# Autodesk Inventor assembly: BG101_trajan20_22
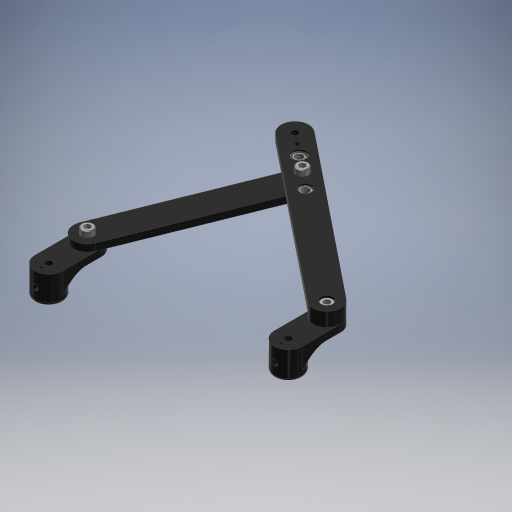
[picture p0: Inventor's stored thumbnail of the model, 512x512]
Saved by Autodesk Inventor 2023 (Build 270158000, 158)
## iProperties
Company: HTBLA Kaindorf
RuleStatus: InUse
Created: 2022-11-06
Part Number: BG101_trajan20_22
Project: Zeichenmaschine_neu
Material: Generisch
Description: Gelenke
Document SubType Name: Assembly
Designer: trajan20
AfterDocNew0: iProperties-Editor_aufrufen
Author: jan
Keywords: 2022
## Documents named in this file (9)
- C:\Users\jan\Documents\Zeichenmaschine_neu\BG101_trajan20_22_Zeichenmaschine_neu_Gelenke.iam
- C:\Users\jan\Documents\Zeichenmaschine_neu\BT301_trajan20_21_Zeichenmaschine_v2_gelenk 1.ipt
- C:\Users\jan\Documents\Zeichenmaschine_neu\BT301_trajan20_21_Zeichenmaschine_v2_gelenk a.ipt
- C:\Users\jan\Documents\Zeichenmaschine_neu\BT303_trajan20_21_Zeichenmaschine_v2_gelenk b.ipt
- C:\Users\jan\Documents\Zeichenmaschine_neu\eigene Normteile\DIN 625 SKF - SKF 628_5-2Z_5x10x4.ipt
- C:\Users\jan\Documents\Zeichenmaschine_neu\Normteile\de-DE\ISO 4762(2)\ISO 4762 - M5 x 16ISO.ipt
- C:\Users\jan\Documents\Zeichenmaschine_neu\Normteile\de-DE\ISO 10511\ISO 10511 - M5.ipt
- C:\Users\jan\Documents\Zeichenmaschine_neu\Normteile\de-DE\DIN 916\DIN 916 - M4  x  10.ipt
- C:\Users\jan\Documents\Zeichenmaschine_neu\BT004_trajan20_22_Zeichenmaschine_neu_QuadratMutter.ipt
## Components (19 placed, 8 different names)
1. BT301_trajan20_21_Zeichenmaschine_v2_gelenk 1:1 — Fluchtend:1, Passend:18, Passend:19, Passend:32, Passend:35, Passend:40, Passend:43, Winkel:1, Passend:45, Passend:46
2. BT301_trajan20_21_Zeichenmaschine_v2_gelenk 1:2 — Fluchtend:1, Passend:4, Passend:5, Passend:30, Passend:37, Passend:41, Passend:43, Winkel:2, Passend:47, Passend:48
3. BT301_trajan20_21_Zeichenmaschine_v2_gelenk a:1 — Passend:18, Passend:19, Passend:20, Passend:21, Passend:22, Passend:34
4. BT303_trajan20_21_Zeichenmaschine_v2_gelenk b:1 — Passend:4, Passend:5, Passend:8, Passend:9, Passend:10, Passend:11, Passend:12, Passend:13, Passend:16, Passend:17, Passend:44
5. BT004_trajan20_22_Zeichenmaschine_neu_QuadratMutter:1 — Winkel:1, Passend:45, Passend:46
6. BT004_trajan20_22_Zeichenmaschine_neu_QuadratMutter:2 — Winkel:2, Passend:47, Passend:48
7. DIN 625 SKF- beidseitig abgedeckt SKF 628/5-2Z:1 — Passend:8, Passend:9
8. DIN 625 SKF- beidseitig abgedeckt SKF 628/5-2Z:2 — Passend:10, Passend:11, Passend:22, Passend:25, Passend:26
9. DIN 625 SKF- beidseitig abgedeckt SKF 628/5-2Z:3 — Passend:12, Passend:13
10. DIN 625 SKF- beidseitig abgedeckt SKF 628/5-2Z:4 — Passend:20, Passend:21, Passend:23, Passend:24
11. DIN 625 SKF- beidseitig abgedeckt SKF 628/5-2Z:5 — Passend:16, Passend:17, Passend:27, Passend:28
12. ISO 4762 M5 x 16:1 — Passend:23, Passend:24, Passend:31, Passend:44
13. ISO 4762 M5 x 16:2 — Passend:25, Passend:26, Passend:33
14. ISO 4762 M5 x 16:3 — Passend:27, Passend:28, Passend:29
15. DIN EN ISO 10511 M5:1 — Passend:29, Passend:30
16. DIN EN ISO 10511 M5:2 — Passend:31, Passend:32
17. DIN EN ISO 10511 M5:3 — Passend:33, Passend:34
18. DIN 916 M4  x  10:1 — Passend:35, Passend:40
19. DIN 916 M4  x  10:3 — Passend:37, Passend:41
## Relationships (40: Mate 37, Angle 2, Flush 1)
- Fluchtend:1 [Flush]: BT301_trajan20_21_Zeichenmaschine_v2_gelenk 1:1 ↔ BT301_trajan20_21_Zeichenmaschine_v2_gelenk 1:2
- Passend:4 [Mate]: BT301_trajan20_21_Zeichenmaschine_v2_gelenk 1:2 ↔ BT303_trajan20_21_Zeichenmaschine_v2_gelenk b:1
- Passend:5 [Mate]: BT301_trajan20_21_Zeichenmaschine_v2_gelenk 1:2 ↔ BT303_trajan20_21_Zeichenmaschine_v2_gelenk b:1
- Passend:8 [Mate]: BT303_trajan20_21_Zeichenmaschine_v2_gelenk b:1 ↔ DIN 625 SKF- beidseitig abgedeckt SKF 628/5-2Z:1
- Passend:9 [Mate]: BT303_trajan20_21_Zeichenmaschine_v2_gelenk b:1 ↔ DIN 625 SKF- beidseitig abgedeckt SKF 628/5-2Z:1
- Passend:10 [Mate]: BT303_trajan20_21_Zeichenmaschine_v2_gelenk b:1 ↔ DIN 625 SKF- beidseitig abgedeckt SKF 628/5-2Z:2
- Passend:11 [Mate]: BT303_trajan20_21_Zeichenmaschine_v2_gelenk b:1 ↔ DIN 625 SKF- beidseitig abgedeckt SKF 628/5-2Z:2
- Passend:12 [Mate]: BT303_trajan20_21_Zeichenmaschine_v2_gelenk b:1 ↔ DIN 625 SKF- beidseitig abgedeckt SKF 628/5-2Z:3
- Passend:13 [Mate]: BT303_trajan20_21_Zeichenmaschine_v2_gelenk b:1 ↔ DIN 625 SKF- beidseitig abgedeckt SKF 628/5-2Z:3
- Passend:16 [Mate]: BT303_trajan20_21_Zeichenmaschine_v2_gelenk b:1 ↔ DIN 625 SKF- beidseitig abgedeckt SKF 628/5-2Z:5
- Passend:17 [Mate]: BT303_trajan20_21_Zeichenmaschine_v2_gelenk b:1 ↔ DIN 625 SKF- beidseitig abgedeckt SKF 628/5-2Z:5
- Passend:18 [Mate]: BT301_trajan20_21_Zeichenmaschine_v2_gelenk 1:1 ↔ BT301_trajan20_21_Zeichenmaschine_v2_gelenk a:1
- Passend:19 [Mate]: BT301_trajan20_21_Zeichenmaschine_v2_gelenk 1:1 ↔ BT301_trajan20_21_Zeichenmaschine_v2_gelenk a:1
- Passend:20 [Mate]: BT301_trajan20_21_Zeichenmaschine_v2_gelenk a:1 ↔ DIN 625 SKF- beidseitig abgedeckt SKF 628/5-2Z:4
- Passend:21 [Mate]: BT301_trajan20_21_Zeichenmaschine_v2_gelenk a:1 ↔ DIN 625 SKF- beidseitig abgedeckt SKF 628/5-2Z:4
- Passend:22 [Mate]: BT301_trajan20_21_Zeichenmaschine_v2_gelenk a:1 ↔ DIN 625 SKF- beidseitig abgedeckt SKF 628/5-2Z:2
- Passend:23 [Mate]: DIN 625 SKF- beidseitig abgedeckt SKF 628/5-2Z:4 ↔ ISO 4762 M5 x 16:1
- Passend:24 [Mate]: DIN 625 SKF- beidseitig abgedeckt SKF 628/5-2Z:4 ↔ ISO 4762 M5 x 16:1
- Passend:25 [Mate]: DIN 625 SKF- beidseitig abgedeckt SKF 628/5-2Z:2 ↔ ISO 4762 M5 x 16:2
- Passend:26 [Mate]: DIN 625 SKF- beidseitig abgedeckt SKF 628/5-2Z:2 ↔ ISO 4762 M5 x 16:2
- Passend:27 [Mate]: DIN 625 SKF- beidseitig abgedeckt SKF 628/5-2Z:5 ↔ ISO 4762 M5 x 16:3
- Passend:28 [Mate]: DIN 625 SKF- beidseitig abgedeckt SKF 628/5-2Z:5 ↔ ISO 4762 M5 x 16:3
- Passend:29 [Mate]: ISO 4762 M5 x 16:3 ↔ DIN EN ISO 10511 M5:1
- Passend:30 [Mate]: BT301_trajan20_21_Zeichenmaschine_v2_gelenk 1:2 ↔ DIN EN ISO 10511 M5:1
- Passend:31 [Mate]: ISO 4762 M5 x 16:1 ↔ DIN EN ISO 10511 M5:2
- Passend:32 [Mate]: BT301_trajan20_21_Zeichenmaschine_v2_gelenk 1:1 ↔ DIN EN ISO 10511 M5:2
- Passend:33 [Mate]: ISO 4762 M5 x 16:2 ↔ DIN EN ISO 10511 M5:3
- Passend:34 [Mate]: BT301_trajan20_21_Zeichenmaschine_v2_gelenk a:1 ↔ DIN EN ISO 10511 M5:3
- Passend:35 [Mate]: BT301_trajan20_21_Zeichenmaschine_v2_gelenk 1:1 ↔ DIN 916 M4  x  10:1
- Passend:37 [Mate]: BT301_trajan20_21_Zeichenmaschine_v2_gelenk 1:2 ↔ DIN 916 M4  x  10:3
- Passend:40 [Mate]: BT301_trajan20_21_Zeichenmaschine_v2_gelenk 1:1 ↔ DIN 916 M4  x  10:1
- Passend:41 [Mate]: BT301_trajan20_21_Zeichenmaschine_v2_gelenk 1:2 ↔ DIN 916 M4  x  10:3
- Passend:43 [Mate] (140 mm): BT301_trajan20_21_Zeichenmaschine_v2_gelenk 1:1 ↔ BT301_trajan20_21_Zeichenmaschine_v2_gelenk 1:2
- Passend:44 [Mate] (140 mm): BT303_trajan20_21_Zeichenmaschine_v2_gelenk b:1 ↔ ISO 4762 M5 x 16:1
- Winkel:1 [Angle] (0 deg): BT301_trajan20_21_Zeichenmaschine_v2_gelenk 1:1 ↔ BT004_trajan20_22_Zeichenmaschine_neu_QuadratMutter:1
- Passend:45 [Mate]: BT301_trajan20_21_Zeichenmaschine_v2_gelenk 1:1 ↔ BT004_trajan20_22_Zeichenmaschine_neu_QuadratMutter:1
- Passend:46 [Mate]: BT301_trajan20_21_Zeichenmaschine_v2_gelenk 1:1 ↔ BT004_trajan20_22_Zeichenmaschine_neu_QuadratMutter:1
- Winkel:2 [Angle] (0 deg): BT301_trajan20_21_Zeichenmaschine_v2_gelenk 1:2 ↔ BT004_trajan20_22_Zeichenmaschine_neu_QuadratMutter:2
- Passend:47 [Mate]: BT301_trajan20_21_Zeichenmaschine_v2_gelenk 1:2 ↔ BT004_trajan20_22_Zeichenmaschine_neu_QuadratMutter:2
- Passend:48 [Mate]: BT301_trajan20_21_Zeichenmaschine_v2_gelenk 1:2 ↔ BT004_trajan20_22_Zeichenmaschine_neu_QuadratMutter:2
